# Autodesk Inventor assembly: Assembly2
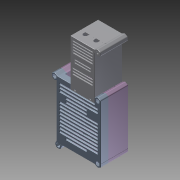
[picture p0: Inventor's stored thumbnail of the model, 180x180]
Saved by Autodesk Inventor 2012 (Build 160160000, 160)
## iProperties
Created: 2018-03-05
Part Number: Assembly2
Document SubType Name: Assembly
Designer: kanu
Author: kanu
## Documents named in this file (6)
- C:\Users\kanu\Documents\Inventor\mi-streamer-box\Assembly2.iam
- C:\Users\kanu\Documents\Inventor\mi-streamer-box\audio case base v2.ipt
- C:\Users\kanu\Documents\Inventor\mi-streamer-box\case add on sdr botom.ipt
- C:\Users\kanu\Documents\Inventor\mi-streamer-box\audio case botom v2.ipt
- C:\Users\kanu\Documents\Inventor\mi-streamer-box\audio case top v3.ipt
- C:\Users\kanu\Documents\Inventor\mi-streamer-box\case add on sdr top v3.ipt
## Components (5 placed, 5 different names)
1. audio case base v2:1 — Mate:1, Mate:2, Mate:3, Insert:1, Insert:2
2. case add on sdr botom:1 — Mate:1, Mate:2, Mate:3, Insert:5, Mate:4
3. audio case botom v2:1 — Insert:1, Insert:2, Insert:3, Insert:4
4. audio case top v3:1 — Insert:3, Insert:4
5. case add on sdr top v3:1 — Insert:5, Mate:4
## Relationships (9: Insert 5, Mate 4)
- Mate:1: audio case base v2:1 ↔ case add on sdr botom:1
- Mate:2: audio case base v2:1 ↔ case add on sdr botom:1
- Mate:3 (0.1 mm): audio case base v2:1 ↔ case add on sdr botom:1
- Insert:1: audio case base v2:1 ↔ audio case botom v2:1
- Insert:2: audio case base v2:1 ↔ audio case botom v2:1
- Insert:3: audio case botom v2:1 ↔ audio case top v3:1
- Insert:4: audio case botom v2:1 ↔ audio case top v3:1
- Insert:5: case add on sdr botom:1 ↔ case add on sdr top v3:1
- Mate:4: case add on sdr botom:1 ↔ case add on sdr top v3:1
